# Autodesk Inventor assembly: GearBox
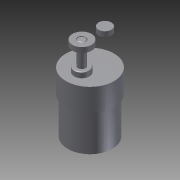
[picture p0: Inventor's stored thumbnail of the model, 180x180]
Saved by Autodesk Inventor 2012 (Build 160160000, 160)
## iProperties
Created: 2011-10-22
Part Number: GearBox
Document SubType Name: Assembly
Designer: KuttaA
Author: KuttaA
## Documents named in this file (3)
- C:\Users\KuttaA\Dropbox\Hexapod Research\Leg Design\Other Parts\GearBox.iam
- C:\Users\KuttaA\Dropbox\Hexapod Research\Leg Design\Other Parts\Motor.ipt
- C:\Users\KuttaA\Dropbox\Hexapod Research\Leg Design\Other Parts\InputGear.ipt
## Components (2 placed, 2 different names)
1. Motor:1 — Flush:1
2. InputGear:1 — Flush:1
## Relationships (1: Flush 1)
- Flush:1: Motor:1 ↔ InputGear:1
